# Autodesk Inventor assembly: BELT_TENSIONER_ASM
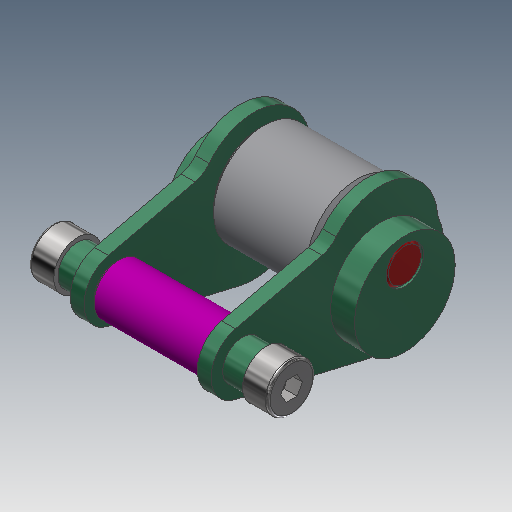
[picture p0: Inventor's stored thumbnail of the model, 512x512]
Saved by Autodesk Inventor 2019.4 (Build 234330000, 330)
## iProperties
Created: 2019-11-13
Part Number: BELT_TENSIONER_ASM
Material: 一般
Document SubType Name: Assembly
Designer: y6tada
Mass: 1.00027 g
Surface Area: 25.1172 cm^2
Volume: 1.00027 cm^3
Density: 1 g/cm^3
Author: y6tada
## Documents named in this file (8)
- C:\Workspace\Yuni9\Inventor\Asm\UPPER_LEG\BELT_TENSIONER_ASM.iam
- C:\Workspace\Yuni9\Inventor\Asm\UPPER_LEG\UPPER_LEG_BELT_TENSIONER.ipt
- C:\Workspace\Yuni9\Inventor\Asm\UPPER_LEG\UPPER_LEG_BELT_TENSIONER_MIR.ipt
- C:\Workspace\Yuni9\Inventor\Asm\UPPER_LEG\BELT_SUPPORT_OUTER.ipt
- C:\Workspace\Yuni9\Inventor\Libs\NSK Bearing\NSK_RB_MF63ZZ\MF63ZZ.iam
- C:\Workspace\Yuni9\Inventor\Libs\SPACER\ARL-2009E.ipt
- C:\Workspace\Yuni9\Inventor\Libs\SHAFT\D3-L15.ipt
- C:\Users\y6tada\Documents\Inventor\Content Center Files\R2019\ja-JP\ISO 4762(2)\ISO 4762 - M2 x 6ISO.ipt
## Components (9 placed, 7 different names)
1. UPPER_LEG_BELT_TENSIONER:1 — フラッシュ:1, フラッシュ:2, メイト:11, メイト:13, メイト:15, フラッシュ:9, メイト:18, メイト:19, メイト:20, 挿入:1
2. UPPER_LEG_BELT_TENSIONER_MIR:1 — メイト:12, メイト:19, メイト:20, 挿入:2
3. BELT_SUPPORT_OUTER:1 — メイト:8, フラッシュ:6, フラッシュ:7, メイト:16, フラッシュ:10
4. MF63ZZ:1 [sub-assembly] — メイト:8, フラッシュ:6, メイト:13, メイト:17
5. ARL-2009E:1 — メイト:11, メイト:12, メイト:18
6. D3-L15:1 — メイト:15, フラッシュ:9, メイト:17
7. MF63ZZ:2 [sub-assembly] — メイト:16, フラッシュ:10
8. ISO 4762 M2 x 6:1 — 挿入:1
9. ISO 4762 M2 x 6:2 — 挿入:2
## Relationships (18: Mate 10, Flush 6, Insert 2)
- フラッシュ:1 [Flush]: UPPER_LEG_BELT_TENSIONER:1
- フラッシュ:2 [Flush]: UPPER_LEG_BELT_TENSIONER:1
- メイト:8 [Mate]: BELT_SUPPORT_OUTER:1 ↔ MF63ZZ:1
- フラッシュ:6 [Flush]: BELT_SUPPORT_OUTER:1 ↔ MF63ZZ:1
- メイト:11 [Mate]: UPPER_LEG_BELT_TENSIONER:1 ↔ ARL-2009E:1
- メイト:12 [Mate]: UPPER_LEG_BELT_TENSIONER_MIR:1 ↔ ARL-2009E:1
- フラッシュ:7 [Flush]: BELT_SUPPORT_OUTER:1
- メイト:13 [Mate] (0.5 mm): UPPER_LEG_BELT_TENSIONER:1 ↔ MF63ZZ:1
- メイト:15 [Mate]: UPPER_LEG_BELT_TENSIONER:1 ↔ D3-L15:1
- フラッシュ:9 [Flush]: UPPER_LEG_BELT_TENSIONER:1 ↔ D3-L15:1
- メイト:16 [Mate]: BELT_SUPPORT_OUTER:1 ↔ MF63ZZ:2
- フラッシュ:10 [Flush]: BELT_SUPPORT_OUTER:1 ↔ MF63ZZ:2
- メイト:17 [Mate]: MF63ZZ:1 ↔ D3-L15:1
- メイト:18 [Mate]: UPPER_LEG_BELT_TENSIONER:1 ↔ ARL-2009E:1
- メイト:19 [Mate]: UPPER_LEG_BELT_TENSIONER:1 ↔ UPPER_LEG_BELT_TENSIONER_MIR:1
- メイト:20 [Mate]: UPPER_LEG_BELT_TENSIONER:1 ↔ UPPER_LEG_BELT_TENSIONER_MIR:1
- 挿入:1 [Insert]: UPPER_LEG_BELT_TENSIONER:1 ↔ ISO 4762 M2 x 6:1
- 挿入:2 [Insert]: UPPER_LEG_BELT_TENSIONER_MIR:1 ↔ ISO 4762 M2 x 6:2
